# Autodesk Inventor assembly: Geared_Servo
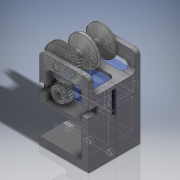
[picture p0: Inventor's stored thumbnail of the model, 180x180]
Saved by Autodesk Inventor 2019 (Build 230136000, 136)
## iProperties
Created: 2020-07-29
Part Number: Geared_Servo
Document SubType Name: Assembly
Designer: Ian
Author: Ian
## Documents named in this file (6)
- C:\Users\Ian\Documents\Pi_Home\Geared_Servo.iam
- D:\Users\Ian\Downloads\Servo.ipt
- C:\Users\Ian\Documents\Pi_Home\Part10.ipt
- C:\Users\Ian\Documents\Pi_Home\Geared_Servo\Design Accelerator\Spur Gears4.iam
- C:\Users\Ian\Documents\Pi_Home\bracket.ipt
- C:\Users\Ian\Documents\Pi_Home\Bracket 2.ipt
## Components (5 placed, 5 different names)
1. Servo:1 — Flush:1, Flush:2, Flush:3, Flush:4, Flush:5
2. Part10:1 — Flush:1
3. Spur Gears:1 [sub-assembly] — Flush:7
4. bracket:1 — Flush:2, Flush:3
5. Bracket 2:1 — Flush:4, Flush:5, Flush:7
## Relationships (6: Flush 6)
- Flush:1: Servo:1 ↔ Part10:1
- Flush:2: Servo:1 ↔ bracket:1
- Flush:3: Servo:1 ↔ bracket:1
- Flush:4: Servo:1 ↔ Bracket 2:1
- Flush:5: Servo:1 ↔ Bracket 2:1
- Flush:7 (0.15 mm): Spur Gears:1 ↔ Bracket 2:1
